# Autodesk Inventor assembly: WhinchFullNM
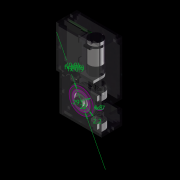
[picture p0: Inventor's stored thumbnail of the model, 180x180]
Saved by Autodesk Inventor 2019 (Build 230136000, 136)
## iProperties
Created: 2019-05-08
Part Number: WhinchFullNM
Document SubType Name: Assembly
Designer: super pig
Author: super pig
## Documents named in this file (19)
- I:\FILES\School\12\DE\Projects\FinalProject\CAD\ShoeWinch\WhinchFullNM.iam
- I:\FILES\School\12\DE\Projects\FinalProject\CAD\ShoeWinch\BaseNM.ipt
- I:\FILES\School\12\DE\Projects\FinalProject\CAD\ShoeWinch\PartsNM.iam
- I:\FILES\School\12\DE\Projects\FinalProject\CAD\ShoeWinch\SideLeftTopNM.ipt
- I:\FILES\School\12\DE\Projects\FinalProject\CAD\ShoeWinch\SideLeftLower.ipt
- I:\FILES\School\12\DE\Projects\FinalProject\CAD\ShoeWinch\SideRightNM.ipt
- I:\FILES\School\12\DE\Projects\FinalProject\CAD\ShoeWinch\SideTopNM.ipt
- I:\FILES\School\12\DE\Projects\FinalProject\CAD\ShoeWinch\SideBottomNM.ipt
- I:\FILES\School\12\DE\Projects\FinalProject\CAD\ShoeWinch\SideFaceTopNM.ipt
- I:\FILES\School\12\DE\Projects\FinalProject\CAD\ShoeWinch\SideFaceBottomNM.ipt
- I:\FILES\School\12\DE\Projects\FinalProject\CAD\ShoeWinch\MotorNM.ipt
- I:\FILES\School\12\DE\Projects\FinalProject\CAD\ShoeWinch\Bearing(8mm).ipt
- I:\FILES\School\12\DE\Projects\FinalProject\CAD\ShoeWinch\Bearing(608).ipt
- I:\FILES\School\12\DE\Projects\FinalProject\CAD\ShoeWinch\LimitSwitch.ipt
- I:\FILES\School\12\DE\Projects\FinalProject\CAD\ShoeWinch\Part3.ipt
- I:\FILES\School\12\DE\Projects\FinalProject\CAD\ShoeWinch\Winch\Design Accelerator\Shaft2.iam
- I:\FILES\School\12\DE\Projects\FinalProject\CAD\ShoeWinch\Winch\Design Accelerator\Spur Gears2.iam
- I:\FILES\School\12\DE\Projects\FinalProject\CAD\ShoeWinch\Winch\Design Accelerator\Worm Gears2.iam
- C:\Users\super pig\Documents\EAGLE\projects\TieMeShoes\selflace.brd.iam
## Components (19 placed, 18 different names)
1. BaseNM:1 — Flush:1, Flush:2, Flush:3, Mate:1, Flush:4, Angle:1, Flush:5, Flush:6, Flush:7, Flush:8, Flush:9
2. PartsNM:1 [sub-assembly] — Mate:1, Flush:4, Angle:1, Mate:8, Mate:10, Flush:13, Mate:11, Flush:14, Mate:12, Mate:14, Mate:17, Mate:18, Mate:19, Mate:20, Mate:22, Mate:23, Mate:24, Flush:16, Flush:17, Mate:26
3. SideLeftTopNM:1 — Flush:5
4. SideLeftLower:1 — Flush:6
5. SideRightNM:1 — Flush:7
6. SideTopNM:1 — Flush:8, Flush:10
7. SideBottomNM:1 — Flush:9, Flush:11
8. SideFaceTopNM:1 — Flush:10
9. SideFaceBottomNM:1 — Flush:11
10. MotorNM:1 — Mate:8, Flush:12, Mate:9, Mate:23, Mate:24
11. Bearing(8mm):1 — Mate:11, Flush:14
12. Bearing(8mm):2 — Mate:10, Flush:13
13. Bearing(608):1 — Mate:15, Mate:16, Mate:17, Mate:22
14. LimitSwitch:1 — Mate:18, Mate:19, Mate:20
15. Part3:1 — Mate:15, Mate:16, Mate:28
16. Shaft:1 [sub-assembly] — Mate:12, Flush:15, Mate:27, Mate:29, Mate:30
17. Spur Gears:1 [sub-assembly] — Flush:12, Mate:9, Flush:15, Mate:29
18. Worm Gears:1 [sub-assembly] — Mate:14, Mate:27, Mate:28, Mate:30
19. selflace.brd:1 [sub-assembly] — Flush:16, Flush:17, Mate:26
## Relationships (39: Mate 21, Flush 17, Angle 1)
- Flush:1: BaseNM:1
- Flush:2: BaseNM:1
- Flush:3: BaseNM:1
- Mate:1: BaseNM:1 ↔ PartsNM:1
- Flush:4: BaseNM:1 ↔ PartsNM:1
- Angle:1 (0 deg): BaseNM:1 ↔ PartsNM:1
- Flush:5: BaseNM:1 ↔ SideLeftTopNM:1
- Flush:6: BaseNM:1 ↔ SideLeftLower:1
- Flush:7: BaseNM:1 ↔ SideRightNM:1
- Flush:8: BaseNM:1 ↔ SideTopNM:1
- Flush:9: BaseNM:1 ↔ SideBottomNM:1
- Flush:10: SideTopNM:1 ↔ SideFaceTopNM:1
- Flush:11: SideBottomNM:1 ↔ SideFaceBottomNM:1
- Mate:8: PartsNM:1 ↔ MotorNM:1
- Flush:12: MotorNM:1 ↔ Spur Gears:1
- Mate:9: MotorNM:1 ↔ Spur Gears:1
- Mate:10: PartsNM:1 ↔ Bearing(8mm):2
- Flush:13: PartsNM:1 ↔ Bearing(8mm):2
- Mate:11: PartsNM:1 ↔ Bearing(8mm):1
- Flush:14: PartsNM:1 ↔ Bearing(8mm):1
- Mate:12: PartsNM:1 ↔ Shaft:1
- Flush:15: Shaft:1 ↔ Spur Gears:1
- Mate:14: PartsNM:1 ↔ Worm Gears:1
- Mate:15: Bearing(608):1 ↔ Part3:1
- Mate:16: Bearing(608):1 ↔ Part3:1
- Mate:17: PartsNM:1 ↔ Bearing(608):1
- Mate:18: PartsNM:1 ↔ LimitSwitch:1
- Mate:19: PartsNM:1 ↔ LimitSwitch:1
- Mate:20: PartsNM:1 ↔ LimitSwitch:1
- Mate:22: PartsNM:1 ↔ Bearing(608):1
- Mate:23: PartsNM:1 ↔ MotorNM:1
- Mate:24: PartsNM:1 ↔ MotorNM:1
- Flush:16: PartsNM:1 ↔ selflace.brd:1
- Flush:17: PartsNM:1 ↔ selflace.brd:1
- Mate:26: PartsNM:1 ↔ selflace.brd:1
- Mate:27: Shaft:1 ↔ Worm Gears:1
- Mate:28: Part3:1 ↔ Worm Gears:1
- Mate:29: Shaft:1 ↔ Spur Gears:1
- Mate:30: Shaft:1 ↔ Worm Gears:1
